# Autodesk Inventor assembly: extraTallPin
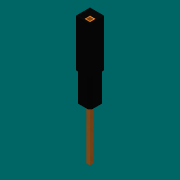
[picture p0: Inventor's stored thumbnail of the model, 180x180]
Saved by Autodesk Inventor 2016 SP1 (Build 200210100, 210)
## iProperties
Created: 2016-04-06
Part Number: extraTallPin
Document SubType Name: Assembly
Designer: sawai
Author: sawai
## Documents named in this file (4)
- C:\Users\sawai\OneDrive\projects\mppcInterface\cad\connector\2.54Header\piExtraTall\extraTallPin.iam
- C:\Users\sawai\OneDrive\projects\mppcInterface\cad\connector\2.54Header\piExtraTall\pinShroud.ipt
- C:\Users\sawai\OneDrive\projects\mppcInterface\cad\connector\2.54Header\piExtraTall\pin.ipt
- C:\Users\sawai\OneDrive\projects\mppcInterface\cad\connector\2.54Header\piExtraTall\spacer.ipt
## Components (4 placed, 3 different names)
1. pinShroud:1 — Mate:6, Flush:7, Flush:8, Mate:7
2. pin:1 — Mate:4, Mate:5, Mate:7
3. spacer:1 — Flush:5, Flush:6, Mate:1, Mate:4, Mate:5, Mate:6, Flush:7, Flush:8
4. spacer:2 — Flush:5, Flush:6, Mate:1
## Relationships (9: Mate 5, Flush 4)
- Flush:5: spacer:1 ↔ spacer:2
- Flush:6: spacer:1 ↔ spacer:2
- Mate:1: spacer:1 ↔ spacer:2
- Mate:4: pin:1 ↔ spacer:1
- Mate:5: pin:1 ↔ spacer:1
- Mate:6: pinShroud:1 ↔ spacer:1
- Flush:7: pinShroud:1 ↔ spacer:1
- Flush:8: pinShroud:1 ↔ spacer:1
- Mate:7: pinShroud:1 ↔ pin:1
